# Autodesk Inventor assembly: Pneumatic Cylindor body
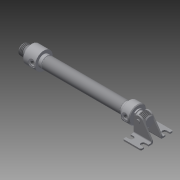
[picture p0: Inventor's stored thumbnail of the model, 180x180]
Saved by Autodesk Inventor 2015 (Build 190159000, 159)
## iProperties
Category: PARTsolutions
Company: BIMBA
Created: 2015-01-25
Part Number: Pneumatic Cylindor body
Catalog Web Link: www.cadenas.de
Description: Original Line Standard Air Cylinders-
Vendor: BIMBA
Document SubType Name: Assembly
Designer: whitaus15
Manufacturer: BIMBA
PSOL_IDENT_0: {$CADENAS_DATA\23d-libs\bimba\bimba\bimba_imperial\bimba_full_line\original_line_cylinders\standard_
PSOL_IDENT_1: air_cylinders\standard_air_cylinder_asmtab.prj},332 {VTYP=3D},{STYP=ASSTAB},{NB=012.5-DP(D-780)(F,D-
PSOL_IDENT_2: 850)},{LINA=012.5-DP},{NN=Original Line Standard Air Cylinders},{DATE=08.09.2014 04:47:41},{GEOMDATE=
PSOL_IDENT_3: 08.09.2014 04:47:39},{VERSION=},{LINEID=30},{LINESUBID=-1},{WBVAR=STROKE,ACTING,MNT,DER,NR,BM,CO,OO,
PSOL_IDENT_4: VO,M,EE,EEL,K,Q,Y,G,T,B,H,SER,SR,NT,W,HL,STPT1,STPT2,STPT3,STPT4,MB,PB,PRC,TB,MN}  {NB=012.5-DP(D-78
PSOL_IDENT_5: 0)(F,D-850)},{LINA=012.5-DP},{KT=DUMMY},{PN=012.5-DP},{PNC=012.5-DP(D-780)(F,D-850)},{PNA=(D-780)(D-
PSOL_IDENT_6: 850)},{DASH=-},{BORE1=0.43750000},{BORE=7/16\" (01)},{BOREPN=01},{STROKE=2.500},{STROKEALG=[0.011:50
PSOL_IDENT_7: /0.001]},{STROKE1=2.500},{ACTING=D},{ACTINGALG= '' , 'Single Acting (SA)' , 'R' , 'Reverse Single Ac
PSOL_IDENT_8: ting (SA)' , 'D' , 'Double Acting (SA)' },{ACTINGPN=D},{MNT=P},{MNTALG= '' , 'Front Nose Mounting (S
PSOL_IDENT_9: A)' , 'P' , 'Rear Pivot Mounting (SA)' , 'X' , 'Double End Mounting (SA)' , 'BF' , 'Front Block Moun
PSOL_IDENT_10: ting (SA)' , 'BR' , 'Rear Block Mounting for Vertical Positioning (SA)' , 'BFT' , 'Front Block Trunn
PSOL_IDENT_11: ion Mounting (SA)' , 'BRT' , 'Rear Block Trunnion Mounting (SA)' },{TYPE=},{MNTPN=P},{DER=},{DERALG=
PSOL_IDENT_12: '' , 'N/A' },{NR=},{NRALG= '' , 'N/A' },{NRPN=},{BM=},{BMALG= '' , 'N/A' },{BMPN=},{CO=},{COALG= ''
PSOL_IDENT_13: , 'N/A' },{OO=},{OOALG= '', 'N/A' },{OOPN=},{VO=Z},{VOALG= 'Z' , 'N/A' },{VOPN=},{OOVOPN=},{M=},{MA
PSOL_IDENT_14: LG= '', 'Without Magnet', 'M', 'With Magnet' },{EE=},{EEL=0.000},{EEMAX=47.5000},{EEALG= '', 'Withou
PSOL_IDENT_15: t Extra Extension', 'EE', 'With Extra Extension' },{EELALG=0},{EEPN=},{EEPN1=0.000},{K=},{KALG= '', '
PSOL_IDENT_16: Standard' , 'K' , 'Ports Rotated 90deg K' },{KPN=},{Q=},{QALG= '' , 'N/A' },{QPN=},{Y=},{YALG= '' , '
PSOL_IDENT_17: Without Pivot Bushing' , 'Y' , 'With Pivot Bushing' },{YPN=},{YCON=},{F=},{FALG= '', 'Non-Coated (St
PSOL_IDENT_18: andard)', 'F', 'Molycoated' },{FPN=},{G=},{GPN=},{GPN99=},{T=},{TALG= '' , 'Standard -20° to 200°F (
PSOL_IDENT_19: -29° to 95°C)' , 'N' , 'Low Temperature' , 'V' , 'High Temperature' },{NPN=},{VPN=},{B=},{BALG= '', '
PSOL_IDENT_20: W/out Bumpers' , 'B' , 'W/ Bumpers' },{BPN=},{H=},{HALG= '', 'N/A' },{HPN=},{SER=},{SERALG= '' , 'Wi
PSOL_IDENT_21: thout Spring Extend/Return' , 'JS' , 'With Spring Return' , 'JR' , 'With Spring Extend' },{SR=},{SRA
PSOL_IDENT_22: LG= '' , 'Standard Stainless Steel' },{SRPN=},{SRCON=0},{NT=},{NTPN=},{W=},{WALG= '' , 'Without Wipe
PSOL_IDENT_23: r' , 'W' , 'With Wiper' },{WPN=},{E=},{EALG= '' , 'Standard Seals/Lube' , 'E' , 'Non-Lube Seals/Lube'
PSOL_IDENT_24: },{EPN=},{HL=},{HLALG= '' , 'Without Low Pressure Hydraulic' , 'HL' , 'With Low Pressure Hydraulic'
PSOL_IDENT_25: },{ST=},{STALG= '' , 'N/A' },{STPT1=},{STPT1ALG= '' , 'N/A' },{STPT2=},{STPT2ALG= '' , 'N/A' },{STP
PSOL_IDENT_26: T3=},{STPT3ALG= '' , 'N/A' },{STPT4=},{STPT4ALG= '' , 'N/A' },{STPN=},{MB=},{MBALG= '' , 'N/A' },{MB
PSOL_IDENT_27: PN=},{MBPNALL=},{MBPNALLREAR=},{PB=D-780},{PBALG= '' , 'Without Pivot Bracket' , 'D-780' , 'D-780' }
PSOL_IDENT_28: ,{PBPN=(D-780)},{PBPNALL=D-780},{PRC=F,D-850},{PRCALG= '' , 'W/out Pivot Rod Clevis' , 'F,D-850' , '
PSOL_IDENT_29: D-850 (front)' },{PRCPN=(F,D-850)},{PRCPNALL=D-850},{TB=},{TBALG= '' , 'N/A' },{TBPN=},{TBPNALL=},{M
PSOL_IDENT_30: N=},{MNALG= '' , 'Without Mounting Nut' , 'F,D-154' , 'D-154 (front)'},{MNPN=},{MNCONF=},{MNCONR=},{
PSOL_IDENT_31: TLEN=3.2700},{FRAC=15.0600},{RGCON=},{RGDACCON=R},{RHCON=P},{RHCON1=P},{RHCONON=1},{RHACCON=R},{FNUT
PSOL_IDENT_32: CON=0},{RNUTCON=0},{FNUTPN=D-154},{RNUTPN=D-154},{FNUTTRANS=0.0000},{RNUTTRANS=0.0000},{VHOLECON=0},
PSOL_IDENT_33: {A1=1.1880},{A1N=0.6880},{A1P=1.1880},{A1B=1.1880},{A4=0.1880},{A4N=0.2500},{A4P=0.1880},{A5=0.0200}
PSOL_IDENT_34: ,{A1H=1.188},{A1NH=0.5000},{A1PH=1.1880},{A1BH=0.8120},{A1SH=0.0000},{A2H=0.1880},{A2NH=0.1880},{LEN
PSOL_IDENT_35: GTH=2.5600},{LENGTH1=2.5600},{LENGTH2=2.6100},{MUL=2.5000},{MUL11=2.5000},{MUL22=7.2},{MUL33=4.7000}
PSOL_IDENT_36: ,{MUL2=2.5000},{MUL211=2.5000},{MUL222=1.4400},{MUL233=0.9400},{SSS=5.0000},{RGLEN=1.0200},{RHLEN=0.
PSOL_IDENT_37: 7700},{SSS1=5.0000},{A13=0.9380},{DIF=0.0000},{G5=0.0000},{ON=0},{SSADD=0.0000},{BADD=0.0000},{MADD=
PSOL_IDENT_38: 0.0000},{NVADD=0.0000},{TRACKL=2.9600},{TRACKCON=D-74168},{TRIMCON=1},{TRIMCON1=0},{PINCON=D-787},{F
PSOL_IDENT_39: SPACE=0.0813},{SPACE=0.0406},{TEXT=0.0711},{S1=0.7500},{D1=0.0000},{D1N=0.4840},{D1B=0.7380},{D1P=0.
PSOL_IDENT_40: 0000},{FA=0.690},{RA=0.6900},{PPATH=standard_air_cylinder_asmtpl.prj},{MATALGHTML=<b>Standard Origin
PSOL_IDENT_41: al Line:</b><dl><dt>Rod:</dt><dd>- Stainless Steel</dd><dd>&nbsp;&nbsp;(5/16 9/16 Bores)</dd><dd>- H
PSOL_IDENT_42: igh Strength Carbon Steel</dd><dd>&nbsp;&nbsp;(3/4 3 Bore)</dd><dd>- Stainless Steel</dd><dd>&nbsp;&
PSOL_IDENT_43: nbsp;(X style DXP/DX/DXDE)</dd><dt>Bearings:</dt><dd>- Sintered Bronze</dd><dt>Body:</dt><dd>- 304 S
PSOL_IDENT_44: tainless Steel</dd><dt>End Caps:</dt><dd>- Aluminum</dd><dt>Seals:</dt><dd>- Buna N</dd></dl>},{ASSC
PSOL_IDENT_45: FGPRA=01DP},{MBPNA=},{MNPNA=},{PRCPNA=(D-850)},{ASSOPTACC=STPT4},{A=5.06},{HADD=0.0000},{WFL=0},{QAD
PSOL_IDENT_46: D=0.000},{QADD1=0.190},{TEST=2.0000},{MNTB=},{STDNUTF=0},{STDNUTR=0}
NN: Original Line Standard Air Cylinders
NT: Standard Male Thread
NB: 012.5-DP(D-780)(F,D-850)
NBSYN: $PNC.
LINA: 012.5-DP
PN: 012.5-DP
PNA: (D-780)(D-850)
BORE: 7/16" [01]
STROKE: 2.500
ACTING: Double [D]
MNT: Rear Pivot [P]
DER: N/A
NR: N/A
BM: N/A
CO: N/A
OO: N/A
VO: N/A
M: Without Magnet Piston
EE: Standard Rod Extension
EEL: 0.000
K: Standard
Q: N/A
Y: Standard Pivot Style
G: Standard Grease Lube
T: Standard -20° to 200°F (-29° to 95°C)
B: Without Bumpers
H: N/A
SER: Without Failsafe Spring Extend/Return
SR: Standard Stainless Steel
W: Without Wiper
HL: Standard 250 PSI Air
STPT1: N/A
STPT2: N/A
STPT3: N/A
STPT4: N/A
MB: N/A
PB: D-780
PRC: D-850 (front)
TB: N/A
MN: Without Mounting Nut
A: 5.06
SUPPLIER: BIMBA
ARTICLENO: 012.5-DP(D-780)(F,D-850)
BOMINFO: 012.5-DP
CREATOR: CADENAS GmbH
Title: 012.5-DP
Author: Cadenas PARTsolutions
## Documents named in this file (10)
- \\lhssvr02\Homedirs\Robotics Club\CAD Model 2015\claw\Actuator end\Pneumatic Cylindor body.iam
- \\lhssvr02\Homedirs\Robotics Club\CAD Model 2015\claw\Actuator end\micros\012_5-DP(D-780)(F,D-850)0000_0_dummy.ipt
- \\lhssvr02\Homedirs\Robotics Club\CAD Model 2015\claw\Actuator end\micros\01R000-0_rod_guide.ipt
- \\lhssvr02\Homedirs\Robotics Club\CAD Model 2015\claw\Actuator end\micros\01R-3_270.ipt
- \\lhssvr02\Homedirs\Robotics Club\CAD Model 2015\claw\Actuator end\micros\01P1000_rear_head.ipt
- \\lhssvr02\Homedirs\Robotics Club\CAD Model 2015\claw\Actuator end\micros\D-787.ipt
- \\lhssvr02\Homedirs\Robotics Club\CAD Model 2015\claw\Actuator end\micros\D-780-dummy.ipt
- \\lhssvr02\Homedirs\Robotics Club\CAD Model 2015\claw\Actuator end\micros\D-9963.ipt
- \\lhssvr02\Homedirs\Robotics Club\CAD Model 2015\claw\Actuator end\micros\D-782.ipt
- \\lhssvr02\Homedirs\Robotics Club\CAD Model 2015\claw\Actuator end\micros\D-850-dummy.ipt
## Components (9 placed, 9 different names)
1. 012_5-DP(D-780)(F,D-850)0000_0_dummy:1 — dummy_XY@1 <-> rod_guide_XY@2, dummy_Z@1 <-> rod_guide_Z@2, dummy_YZ@1 <-> rod_guide_YZ@2
2. 01R000-0_rod_guide:1 — dummy_XY@1 <-> rod_guide_XY@2, dummy_Z@1 <-> rod_guide_Z@2, dummy_YZ@1 <-> rod_guide_YZ@2, to_tube_XY@2 <-> tube_front_XY@3, to_tube_Z@2 <-> tube_front_Z@3, to_tube_YZ@2 <-> tube_front_YZ@3
3. 01R-3_270:1 — to_tube_XY@2 <-> tube_front_XY@3, to_tube_Z@2 <-> tube_front_Z@3, to_tube_YZ@2 <-> tube_front_YZ@3, tube_rear_XY@3 <-> to_tube_XY@4, tube_rear_Z@3 <-> to_tube_Z@4, tube_rear_YZ@3 <-> to_tube_YZ@4
4. 01P1000_rear_head:1 — tube_rear_XY@3 <-> to_tube_XY@4, tube_rear_Z@3 <-> to_tube_Z@4, tube_rear_YZ@3 <-> to_tube_YZ@4, to_pin_XY@4 <-> pin_XY@5, to_pin_Z@4 <-> pin_Z@5, to_pin_YZ@4 <-> pin_YZ@5, to_pin_XY@4 <-> to_cyl_XY@6, to_pin_Z@4 <-> to_cyl_Z@6
5. D-787:1 — to_pin_XY@4 <-> pin_XY@5, to_pin_Z@4 <-> pin_Z@5, to_pin_YZ@4 <-> pin_YZ@5
6. D-780-dummy:1 — to_pin_XY@4 <-> to_cyl_XY@6, to_pin_Z@4 <-> to_cyl_Z@6, to_l_XY@6 <-> to_dummy_L_XY@7, to_l_Z@6 <-> to_dummy_L_Z@7, to_l_YZ@6 <-> to_dummy_L_YZ@7, to_r_XY@6 <-> to_dummy_R_XY@8, to_r_Z@6 <-> to_dummy_R_Z@8, to_r_YZ@6 <-> to_dummy_R_YZ@8
7. D-9963:1 — to_l_XY@6 <-> to_dummy_L_XY@7, to_l_Z@6 <-> to_dummy_L_Z@7, to_l_YZ@6 <-> to_dummy_L_YZ@7
8. D-782:1 — to_r_XY@6 <-> to_dummy_R_XY@8, to_r_Z@6 <-> to_dummy_R_Z@8, to_r_YZ@6 <-> to_dummy_R_YZ@8
9. D-850-dummy:1
## Relationships (20: Mate 8, Flush 6, Angle 6)
- dummy_XY@1 <-> rod_guide_XY@2 [Flush]: 012_5-DP(D-780)(F,D-850)0000_0_dummy:1 ↔ 01R000-0_rod_guide:1
- dummy_Z@1 <-> rod_guide_Z@2 [Mate]: 012_5-DP(D-780)(F,D-850)0000_0_dummy:1 ↔ 01R000-0_rod_guide:1
- dummy_YZ@1 <-> rod_guide_YZ@2 [Angle] (0 deg): 012_5-DP(D-780)(F,D-850)0000_0_dummy:1 ↔ 01R000-0_rod_guide:1
- to_tube_XY@2 <-> tube_front_XY@3 [Flush]: 01R000-0_rod_guide:1 ↔ 01R-3_270:1
- to_tube_Z@2 <-> tube_front_Z@3 [Mate]: 01R000-0_rod_guide:1 ↔ 01R-3_270:1
- to_tube_YZ@2 <-> tube_front_YZ@3 [Angle] (0 deg): 01R000-0_rod_guide:1 ↔ 01R-3_270:1
- tube_rear_XY@3 <-> to_tube_XY@4 [Flush]: 01R-3_270:1 ↔ 01P1000_rear_head:1
- tube_rear_Z@3 <-> to_tube_Z@4 [Mate]: 01R-3_270:1 ↔ 01P1000_rear_head:1
- tube_rear_YZ@3 <-> to_tube_YZ@4 [Angle] (0 deg): 01R-3_270:1 ↔ 01P1000_rear_head:1
- to_pin_XY@4 <-> pin_XY@5 [Mate]: 01P1000_rear_head:1 ↔ D-787:1
- to_pin_Z@4 <-> pin_Z@5 [Mate]: 01P1000_rear_head:1 ↔ D-787:1
- to_pin_YZ@4 <-> pin_YZ@5 [Angle] (0 deg): 01P1000_rear_head:1 ↔ D-787:1
- to_pin_XY@4 <-> to_cyl_XY@6 [Flush]: 01P1000_rear_head:1 ↔ D-780-dummy:1
- to_pin_Z@4 <-> to_cyl_Z@6 [Mate]: 01P1000_rear_head:1 ↔ D-780-dummy:1
- to_l_XY@6 <-> to_dummy_L_XY@7 [Flush]: D-780-dummy:1 ↔ D-9963:1
- to_l_Z@6 <-> to_dummy_L_Z@7 [Mate]: D-780-dummy:1 ↔ D-9963:1
- to_l_YZ@6 <-> to_dummy_L_YZ@7 [Angle] (0 deg): D-780-dummy:1 ↔ D-9963:1
- to_r_XY@6 <-> to_dummy_R_XY@8 [Flush]: D-780-dummy:1 ↔ D-782:1
- to_r_Z@6 <-> to_dummy_R_Z@8 [Mate]: D-780-dummy:1 ↔ D-782:1
- to_r_YZ@6 <-> to_dummy_R_YZ@8 [Angle] (0 deg): D-780-dummy:1 ↔ D-782:1
